# Autodesk Inventor assembly: Capper Assembly
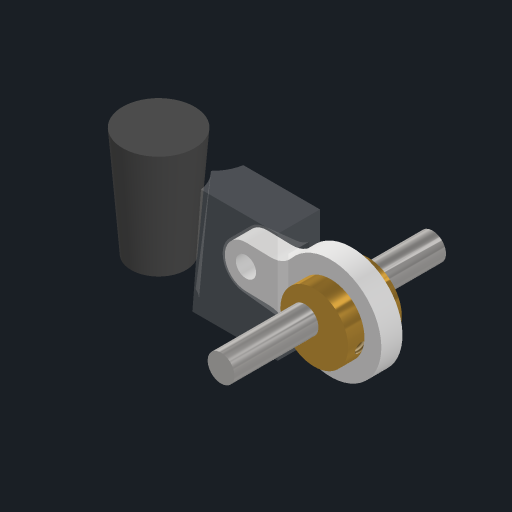
[picture p0: Inventor's stored thumbnail of the model, 512x512]
Saved by Autodesk Inventor 2023.1 (Build 271208000, 208)
## iProperties
Created: 2023-05-23
Part Number: Capper Assembly
Document SubType Name: Assembly
Designer: Jarrett
Author: Jarrett
## Documents named in this file (6)
- C:\Users\Jarrett\Desktop\Projects\BehrendURCMechanical\CAD\Science\Capper Assembly.iam
- C:\Users\Jarrett\Desktop\Projects\BehrendURCMechanical\CAD\Science\Capper Gate Bushing.ipt
- C:\Users\Jarrett\Desktop\Projects\BehrendURCMechanical\CAD\Science\Capper Gate Linkage.ipt
- C:\Users\Jarrett\Desktop\Projects\BehrendURCMechanical\CAD\Science\Capper Gate.ipt
- C:\Users\Jarrett\Desktop\Projects\BehrendURCMechanical\CAD\Science\Capper Gate Shaft.ipt
- C:\Users\Jarrett\Desktop\Projects\BehrendURCMechanical\CAD\Science\SC-1-01-Test Tube Cap.ipt
## Components (5 placed, 5 different names)
1. Capper Gate Bushing:1 — Rotational:2, Flush:1, Mate:1, Mate:3
2. Capper Gate Linkage:1 — Rotational:2, Rotational:3
3. Capper Gate:1 — Mate:2, Rotational:3
4. Capper Gate Shaft:1 — Mate:3
5. SC-1-01-Test Tube Cap:1
## Relationships (6: Mate 3, RevoluteJoint 2, Flush 1)
- Rotational:2 [RevoluteJoint]: Capper Gate Bushing:1 ↔ Capper Gate Linkage:1
- Flush:1: Capper Gate Bushing:1
- Mate:1: Capper Gate Bushing:1
- Mate:2 (-13 mm): Capper Gate:1
- Rotational:3 [RevoluteJoint]: Capper Gate Linkage:1 ↔ Capper Gate:1
- Mate:3: Capper Gate Bushing:1 ↔ Capper Gate Shaft:1
